# Autodesk Inventor assembly: SE cubierta optica
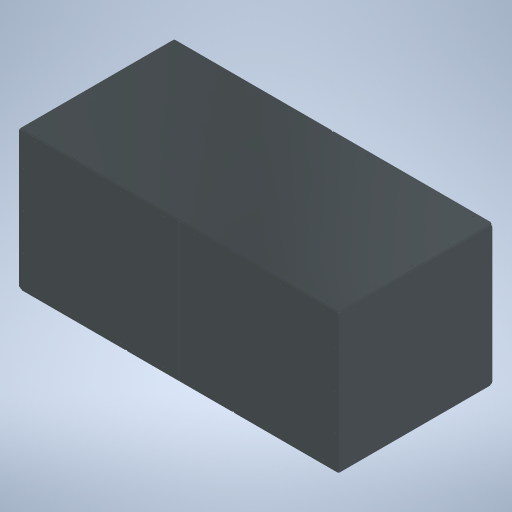
[picture p0: Inventor's stored thumbnail of the model, 512x512]
Saved by Autodesk Inventor 2024.2 (Build 282272000, 272)
## iProperties
Created: 2025-11-13
Part Number: SE cubierta optica
Document SubType Name: Assembly
Designer: ja.restrepo1
Author: ja.restrepo1
## Documents named in this file (5)
- I:\MICROMECANICA\ALTAS ENERGIAS\Deteccion de Muones\Detectores centelladores\Partes Detector Centellador\SE cubierta optica\SE cubierta optica.iam
- I:\MICROMECANICA\ALTAS ENERGIAS\Deteccion de Muones\Detectores centelladores\Partes Detector Centellador\SE cubierta optica\Encerramiento\1000x900.ipt
- I:\MICROMECANICA\ALTAS ENERGIAS\Deteccion de Muones\Detectores centelladores\Partes Detector Centellador\SE cubierta optica\Encerramiento\1040x1000 esquina.ipt
- I:\MICROMECANICA\ALTAS ENERGIAS\Deteccion de Muones\Detectores centelladores\Partes Detector Centellador\SE cubierta optica\Encerramiento\1040x900 esquina.ipt
- I:\MICROMECANICA\ALTAS ENERGIAS\Deteccion de Muones\Detectores centelladores\Partes Detector Centellador\SE cubierta optica\Encerramiento\700x1000.ipt
## Components (12 placed, 4 different names)
1. 700x1000:2 — Nivelación:3, Nivelación:4, Coincidencia:3, Nivelación:5, Nivelación:6, Nivelación:7, Nivelación:8, Coincidencia:4, Nivelación:13
2. 1000x900:1 — Coincidencia:5, Nivelación:10, Coincidencia:6, Nivelación:11, Nivelación:22, Coincidencia:11, Coincidencia:13
3. 1000x900:2 — Coincidencia:8, Nivelación:15, Nivelación:16, Nivelación:25
4. 1040x1000 esquina:1 — Nivelación:5, Nivelación:8, Coincidencia:8, Nivelación:15, Nivelación:24
5. 1040x1000 esquina:2 — Nivelación:6, Nivelación:7, Coincidencia:4, Coincidencia:5, Nivelación:10, Nivelación:12, Coincidencia:13
6. 1040x900 esquina:1 — Coincidencia:7, Nivelación:13, Nivelación:14, Nivelación:16
7. 1040x900 esquina:2 — Coincidencia:6, Nivelación:11, Nivelación:12, Coincidencia:7, Nivelación:14, Coincidencia:10, Nivelación:21
8. 1040x900 esquina:3 — Coincidencia:11, Coincidencia:12, Nivelación:23, Nivelación:26
9. 1040x900 esquina:4 — Coincidencia:12, Nivelación:23, Nivelación:24, Nivelación:25, Nivelación:26
10. 1040x1000 esquina:3 — Nivelación:18, Nivelación:19, Coincidencia:9
11. 1040x1000 esquina:4 — Nivelación:17, Nivelación:20, Coincidencia:10, Nivelación:21, Nivelación:22
12. 700x1000:1 — Nivelación:17, Nivelación:18, Nivelación:19, Nivelación:20, Coincidencia:9
## Relationships (38: Flush 25, Mate 13)
- [Flush]: 1040x1000 esquina:3 ↔ 700x1000:1
- [Mate]: 1040x1000 esquina:4 ↔ 700x1000:1
- [Flush]: 700x1000:2 ↔ 1040x1000 esquina:2
- [Mate]: 700x1000:2 ↔ 1040x1000 esquina:1
- Nivelación:3 [Flush]: 700x1000:2
- Nivelación:4 [Flush]: 700x1000:2
- Coincidencia:3 [Mate] (456 mm): 700x1000:2
- Nivelación:5 [Flush]: 700x1000:2 ↔ 1040x1000 esquina:1
- Nivelación:6 [Flush]: 700x1000:2 ↔ 1040x1000 esquina:2
- Nivelación:7 [Flush]: 700x1000:2 ↔ 1040x1000 esquina:2
- Nivelación:8 [Flush]: 700x1000:2 ↔ 1040x1000 esquina:1
- Coincidencia:4 [Mate]: 700x1000:2 ↔ 1040x1000 esquina:2
- Coincidencia:5 [Mate]: 1000x900:1 ↔ 1040x1000 esquina:2
- Nivelación:10 [Flush]: 1000x900:1 ↔ 1040x1000 esquina:2
- Coincidencia:6 [Mate]: 1000x900:1 ↔ 1040x900 esquina:2
- Nivelación:11 [Flush]: 1000x900:1 ↔ 1040x900 esquina:2
- Nivelación:12 [Flush] (-5 mm): 1040x1000 esquina:2 ↔ 1040x900 esquina:2
- Coincidencia:7 [Mate] (5 mm): 1040x900 esquina:1 ↔ 1040x900 esquina:2
- Nivelación:13 [Flush] (-5 mm): 700x1000:2 ↔ 1040x900 esquina:1
- Nivelación:14 [Flush]: 1040x900 esquina:1 ↔ 1040x900 esquina:2
- Coincidencia:8 [Mate]: 1000x900:2 ↔ 1040x1000 esquina:1
- Nivelación:15 [Flush] (-5 mm): 1000x900:2 ↔ 1040x1000 esquina:1
- Nivelación:16 [Flush]: 1000x900:2 ↔ 1040x900 esquina:1
- Nivelación:17 [Flush]: 1040x1000 esquina:4 ↔ 700x1000:1
- Nivelación:18 [Flush]: 1040x1000 esquina:3 ↔ 700x1000:1
- Nivelación:19 [Flush]: 1040x1000 esquina:3 ↔ 700x1000:1
- Nivelación:20 [Flush]: 1040x1000 esquina:4 ↔ 700x1000:1
- Coincidencia:9 [Mate]: 1040x1000 esquina:3 ↔ 700x1000:1
- Coincidencia:10 [Mate]: 1040x900 esquina:2 ↔ 1040x1000 esquina:4
- Nivelación:21 [Flush]: 1040x900 esquina:2 ↔ 1040x1000 esquina:4
- Nivelación:22 [Flush]: 1000x900:1 ↔ 1040x1000 esquina:4
- Coincidencia:11 [Mate]: 1000x900:1 ↔ 1040x900 esquina:3
- Coincidencia:12 [Mate]: 1040x900 esquina:3 ↔ 1040x900 esquina:4
- Nivelación:23 [Flush]: 1040x900 esquina:3 ↔ 1040x900 esquina:4
- Nivelación:24 [Flush]: 1040x1000 esquina:1 ↔ 1040x900 esquina:4
- Nivelación:25 [Flush]: 1000x900:2 ↔ 1040x900 esquina:4
- Nivelación:26 [Flush]: 1040x900 esquina:3 ↔ 1040x900 esquina:4
- Coincidencia:13 [Mate]: 1000x900:1 ↔ 1040x1000 esquina:2
